# Autodesk Inventor assembly: Robot1
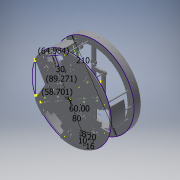
[picture p0: Inventor's stored thumbnail of the model, 180x180]
Saved by Autodesk Inventor 2018 (Build 220112000, 112)
## iProperties
Created: 2017-10-30
Part Number: Robot1
Document SubType Name: Assembly
Designer: BrisbaneMatt
Author: BrisbaneMatt
## Documents named in this file (7)
- C:\Users\matth\git\Robotics-2018\Design and Hardware\mk2\Robot1.iam
- C:\Users\matth\git\Robotics-2018\Design and Hardware\mk2\Base\Base3.ipt
- C:\Users\matth\git\Robotics-2018\Design and Hardware\mk2\Standoff 60mm.ipt
- C:\Users\matth\git\Robotics-2018\Design and Hardware\mk2\Capture Zone\Capture Zone5.ipt
- C:\Users\matth\git\Robotics-2018\Design and Hardware\mk2\Wheel Guards\Wheel Guard1.ipt
- C:\Users\matth\git\Robotics-2018\Design and Hardware\mk2\Standoff 20mm.ipt
- C:\Users\matth\git\Robotics-2018\Design and Hardware\mk2\Tsop Ring-Circuit Board Plate\Tsop Ring-Circuit Board Plate6.ipt
## Components (19 placed, 6 different names)
1. Base3:1 — Mate:1, Mate:2, Mate:3, Mate:4, Mate:5, Mate:6, Mate:7, Mate:9, Mate:10, Mate:11, Mate:12, Mate:13, Mate:14, Mate:15
2. Standoff 60mm:1 — Mate:2
3. Standoff 60mm:2 — Mate:5
4. Standoff 60mm:3 — Mate:1
5. Standoff 60mm:4 — Mate:4
6. Standoff 60mm:5 — Mate:3
7. Standoff 60mm:6 — Mate:9
8. Standoff 60mm:7 — Mate:6
9. Standoff 60mm:9 — Mate:7
10. Capture Zone5:1 — Mate:10, Mate:19, Mate:20
11. Wheel Guard1:1 — Mate:12, Mate:13, Mate:18
12. Wheel Guard1:2 — Mate:14, Mate:15, Mate:16
13. Wheel Guard1:3 — Mate:11, Mate:17
14. Standoff 20mm:1 — Mate:20
15. Standoff 20mm:2 — Mate:16, Mate:21
16. Standoff 20mm:3 — Mate:18
17. Standoff 20mm:4 — Mate:19
18. Standoff 20mm:5 — Mate:17
19. Tsop Ring-Circuit Board Plate6:1 — Mate:21
## Relationships (20: Mate 20)
- Mate:1: Base3:1 ↔ Standoff 60mm:3
- Mate:2: Base3:1 ↔ Standoff 60mm:1
- Mate:3: Base3:1 ↔ Standoff 60mm:5
- Mate:4: Base3:1 ↔ Standoff 60mm:4
- Mate:5: Base3:1 ↔ Standoff 60mm:2
- Mate:6: Base3:1 ↔ Standoff 60mm:7
- Mate:7: Base3:1 ↔ Standoff 60mm:9
- Mate:9: Base3:1 ↔ Standoff 60mm:6
- Mate:10: Base3:1 ↔ Capture Zone5:1
- Mate:11: Base3:1 ↔ Wheel Guard1:3
- Mate:12: Base3:1 ↔ Wheel Guard1:1
- Mate:13: Base3:1 ↔ Wheel Guard1:1
- Mate:14: Base3:1 ↔ Wheel Guard1:2
- Mate:15: Base3:1 ↔ Wheel Guard1:2
- Mate:16: Wheel Guard1:2 ↔ Standoff 20mm:2
- Mate:17: Wheel Guard1:3 ↔ Standoff 20mm:5
- Mate:18: Wheel Guard1:1 ↔ Standoff 20mm:3
- Mate:19: Capture Zone5:1 ↔ Standoff 20mm:4
- Mate:20: Capture Zone5:1 ↔ Standoff 20mm:1
- Mate:21: Standoff 20mm:2 ↔ Tsop Ring-Circuit Board Plate6:1
